# Autodesk Inventor assembly: Donja_konstrinkcija_s_drop_mehanizmom_v.2.0
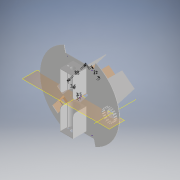
[picture p0: Inventor's stored thumbnail of the model, 180x180]
Saved by Autodesk Inventor 2020 (Build 240168000, 168)
## iProperties
Created: 2020-10-13
Part Number: Donja_konstrinkcija_s_drop_mehanizmom_v.2.0
Document SubType Name: Assembly
Designer: Sičaja
Author: Sičaja
## Documents named in this file (3)
- C:\Users\Sicaja\Documents\Projects\3D Drawings\Inventor_draws\Robocup\Inverntor_parts_for_print\Step_files_for_print\Donja_konstrinkcija_s_drop_mehanizmom_v.2.0.iam
- C:\Users\Sicaja\Documents\Projects\3D Drawings\Inventor_draws\Robocup\Inverntor_parts_for_print\KonstrukcijaDonjiDio_v.1.1.ipt
- C:\Users\Sicaja\Documents\Projects\3D Drawings\Inventor_draws\Robocup\Inverntor_parts_for_print\DropMechanism_v.2.0.ipt
## Components (2 placed, 2 different names)
1. KonstrukcijaDonjiDio_v.1.1:1 — Mate:1, Flush:1, Flush:2
2. DropMechanism_v.2.0:1 — Mate:1, Flush:1, Flush:2
## Relationships (3: Flush 2, Mate 1)
- Mate:1: KonstrukcijaDonjiDio_v.1.1:1 ↔ DropMechanism_v.2.0:1
- Flush:1: KonstrukcijaDonjiDio_v.1.1:1 ↔ DropMechanism_v.2.0:1
- Flush:2: KonstrukcijaDonjiDio_v.1.1:1 ↔ DropMechanism_v.2.0:1
